# Autodesk Inventor assembly: CH-0-01-GearBoxAssembly
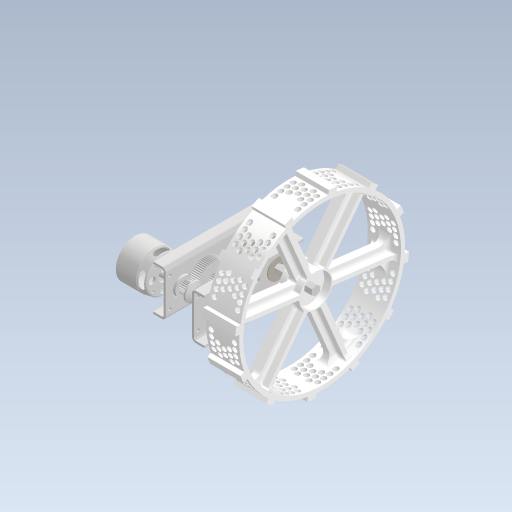
[picture p0: Inventor's stored thumbnail of the model, 512x512]
Saved by Autodesk Inventor 2023 (Build 270158000, 158)
## iProperties
Created: 2022-11-08
Part Number: CH-0-01-GearBoxAssembly
Document SubType Name: Assembly
Designer: Dave
Author: Dave
## Documents named in this file (13)
- C:\Users\Dave\Documents\GitHub\BehrendURCMechanical\CAD\Chassis\GearBox\CH-0-01-GearBoxAssembly.iam
- C:\Users\Dave\Documents\GitHub\BehrendURCMechanical\CAD\Chassis\GearBox\CH-1-01-0.5HexBearing.ipt
- C:\Users\Dave\Documents\GitHub\BehrendURCMechanical\CAD\Chassis\GearBox\CH-1-01-0.25IDSmoothBoreBearing.ipt
- C:\Users\Dave\Documents\GitHub\BehrendURCMechanical\CAD\Chassis\GearBox\CH-1-01-20T_0.5x0.25BoreGear.ipt
- C:\Users\Dave\Documents\GitHub\BehrendURCMechanical\CAD\Chassis\GearBox\CH-1-01-20T_0.5x8mmBoreGear.ipt
- C:\Users\Dave\Documents\GitHub\BehrendURCMechanical\CAD\Chassis\GearBox\CH-1-01-60T_0.5x0.25BoreGear.ipt
- C:\Users\Dave\Documents\GitHub\BehrendURCMechanical\CAD\Chassis\GearBox\Ch-1-01-0.5x4.5HexShaft.ipt
- C:\Users\Dave\Documents\GitHub\BehrendURCMechanical\CAD\Chassis\GearBox\CH-1-01-0.25x1.875SmoothShaft.ipt
- C:\Users\Dave\Documents\GitHub\BehrendURCMechanical\CAD\Chassis\CH-1-03-6SpokeWheel.ipt
- C:\Users\Dave\Documents\GitHub\BehrendURCMechanical\CAD\Chassis\GearBox\Drive Motor Shaft Coupler.ipt
- C:\Users\Dave\Documents\GitHub\BehrendURCMechanical\CAD\Chassis\GearBox\Drive Motor.ipt
- C:\Users\Dave\Documents\GitHub\BehrendURCMechanical\CAD\Chassis\GearBox\CH-1-01-GearboxHousingMotorSide.ipt
- C:\Users\Dave\Documents\GitHub\BehrendURCMechanical\CAD\Chassis\GearBox\CH-1-01-GearboxHousingWheelSide.ipt
## Components (20 placed, 12 different names)
1. CH-1-01-0.5HexBearing:1 — Mate:23, Flush:6, Mate:29, Insert:4, Mate:37
2. CH-1-01-0.5HexBearing:2 — Mate:21, Mate:23, Flush:8, Flush:9, Flush:12, Mate:26, Mate:27, Mate:33, Insert:3
3. CH-1-01-0.25IDSmoothBoreBearing:1 — Mate:18, Flush:9, Flush:11, Mate:25
4. CH-1-01-0.25IDSmoothBoreBearing:2 — Mate:17, Flush:8, Flush:10, Mate:24, Mate:35
5. CH-1-01-0.25IDSmoothBoreBearing:3 — Mate:19, Flush:6, Flush:7
6. CH-1-01-0.25IDSmoothBoreBearing:4 — Mate:16, Flush:7, Mate:36
7. CH-1-01-20T_0.5x0.25BoreGear:1 — Mate:4, Mate:5, Flush:3, Mate:6, Mate:16, Mate:31, Rotation:6
8. CH-1-01-20T_0.5x0.25BoreGear:2 — Mate:7, Mate:8, Mate:10, Mate:19, Angle:16
9. CH-1-01-20T_0.5x8mmBoreGear:1 — Mate:1, Flush:1, Flush:2, Mate:2, Rotation:1, Angle:2, Insert:1
10. CH-1-01-60T_0.5x0.25BoreGear:1 — Flush:3, Mate:6, Mate:7, Mate:8, Mate:18, Rotation:6, Angle:16, Mate:34
11. CH-1-01-60T_0.5x0.25BoreGear:2 — Flush:2, Mate:2, Mate:3, Mate:4, Mate:5, Mate:17, Mate:21, Rotation:1, Mate:31
12. Ch-1-01-0.5x4.5HexShaft:1 — Flush:12, Mate:26, Mate:27, Flush:14, Mate:30
13. CH-1-01-0.25x1.875SmoothShaft:1 — Flush:10, Mate:24
14. CH-1-01-0.25x1.875SmoothShaft:2 — Flush:11, Mate:25
15. CH-1-03-6SpokeWheel:1 — Mate:29, Flush:14, Mate:30
16. CH-1-01-60T_0.5x0.25BoreGear:3 — Mate:33, Mate:34, Mate:37
17. Drive Motor Shaft Coupler:1 — Insert:1, Insert:2
18. Drive Motor:1 — Insert:2
19. CH-1-01-GearboxHousingMotorSide:1 — Insert:3, Mate:35
20. CH-1-01-GearboxHousingWheelSide:1 — Insert:4, Mate:36
## Relationships (47: Mate 27, Flush 12, Insert 4, RelateRotation 2, Angle 2)
- Mate:1: CH-1-01-20T_0.5x8mmBoreGear:1
- Flush:1: CH-1-01-20T_0.5x8mmBoreGear:1
- Flush:2: CH-1-01-20T_0.5x8mmBoreGear:1 ↔ CH-1-01-60T_0.5x0.25BoreGear:2
- Mate:2 (31.75 mm): CH-1-01-20T_0.5x8mmBoreGear:1 ↔ CH-1-01-60T_0.5x0.25BoreGear:2
- Mate:3: CH-1-01-60T_0.5x0.25BoreGear:2
- Mate:4: CH-1-01-20T_0.5x0.25BoreGear:1 ↔ CH-1-01-60T_0.5x0.25BoreGear:2
- Mate:5: CH-1-01-20T_0.5x0.25BoreGear:1 ↔ CH-1-01-60T_0.5x0.25BoreGear:2
- Flush:3: CH-1-01-20T_0.5x0.25BoreGear:1 ↔ CH-1-01-60T_0.5x0.25BoreGear:1
- Mate:6 (31.75 mm): CH-1-01-20T_0.5x0.25BoreGear:1 ↔ CH-1-01-60T_0.5x0.25BoreGear:1
- Mate:7: CH-1-01-20T_0.5x0.25BoreGear:2 ↔ CH-1-01-60T_0.5x0.25BoreGear:1
- Mate:8: CH-1-01-20T_0.5x0.25BoreGear:2 ↔ CH-1-01-60T_0.5x0.25BoreGear:1
- Flush:5
- Mate:10: CH-1-01-20T_0.5x0.25BoreGear:2
- Mate:16: CH-1-01-0.25IDSmoothBoreBearing:4 ↔ CH-1-01-20T_0.5x0.25BoreGear:1
- Mate:17: CH-1-01-0.25IDSmoothBoreBearing:2 ↔ CH-1-01-60T_0.5x0.25BoreGear:2
- Mate:18: CH-1-01-0.25IDSmoothBoreBearing:1 ↔ CH-1-01-60T_0.5x0.25BoreGear:1
- Mate:19: CH-1-01-0.25IDSmoothBoreBearing:3 ↔ CH-1-01-20T_0.5x0.25BoreGear:2
- Mate:21: CH-1-01-0.5HexBearing:2 ↔ CH-1-01-60T_0.5x0.25BoreGear:2
- Mate:23: CH-1-01-0.5HexBearing:1 ↔ CH-1-01-0.5HexBearing:2
- Flush:6: CH-1-01-0.5HexBearing:1 ↔ CH-1-01-0.25IDSmoothBoreBearing:3
- Flush:7: CH-1-01-0.25IDSmoothBoreBearing:3 ↔ CH-1-01-0.25IDSmoothBoreBearing:4
- Flush:8: CH-1-01-0.5HexBearing:2 ↔ CH-1-01-0.25IDSmoothBoreBearing:2
- Flush:9: CH-1-01-0.5HexBearing:2 ↔ CH-1-01-0.25IDSmoothBoreBearing:1
- Flush:10: CH-1-01-0.25IDSmoothBoreBearing:2 ↔ CH-1-01-0.25x1.875SmoothShaft:1
- Mate:24: CH-1-01-0.25IDSmoothBoreBearing:2 ↔ CH-1-01-0.25x1.875SmoothShaft:1
- Flush:11: CH-1-01-0.25IDSmoothBoreBearing:1 ↔ CH-1-01-0.25x1.875SmoothShaft:2
- Mate:25: CH-1-01-0.25IDSmoothBoreBearing:1 ↔ CH-1-01-0.25x1.875SmoothShaft:2
- Flush:12: CH-1-01-0.5HexBearing:2 ↔ Ch-1-01-0.5x4.5HexShaft:1
- Mate:26: CH-1-01-0.5HexBearing:2 ↔ Ch-1-01-0.5x4.5HexShaft:1
- Mate:27: CH-1-01-0.5HexBearing:2 ↔ Ch-1-01-0.5x4.5HexShaft:1
- Mate:29: CH-1-01-0.5HexBearing:1 ↔ CH-1-03-6SpokeWheel:1
- Flush:14: Ch-1-01-0.5x4.5HexShaft:1 ↔ CH-1-03-6SpokeWheel:1
- Mate:30: Ch-1-01-0.5x4.5HexShaft:1 ↔ CH-1-03-6SpokeWheel:1
- Rotation:1 [RelateRotation] (0.3333 ul): CH-1-01-20T_0.5x8mmBoreGear:1 ↔ CH-1-01-60T_0.5x0.25BoreGear:2
- Angle:2 (926 deg): CH-1-01-20T_0.5x8mmBoreGear:1
- Mate:31: CH-1-01-20T_0.5x0.25BoreGear:1 ↔ CH-1-01-60T_0.5x0.25BoreGear:2
- Rotation:6 [RelateRotation] (0.3333 ul): CH-1-01-20T_0.5x0.25BoreGear:1 ↔ CH-1-01-60T_0.5x0.25BoreGear:1
- Angle:16 (0 deg): CH-1-01-20T_0.5x0.25BoreGear:2 ↔ CH-1-01-60T_0.5x0.25BoreGear:1
- Mate:33: CH-1-01-0.5HexBearing:2 ↔ CH-1-01-60T_0.5x0.25BoreGear:3
- Mate:34: CH-1-01-60T_0.5x0.25BoreGear:1 ↔ CH-1-01-60T_0.5x0.25BoreGear:3
- Insert:1: CH-1-01-20T_0.5x8mmBoreGear:1 ↔ Drive Motor Shaft Coupler:1
- Insert:2 (12.7 mm): Drive Motor Shaft Coupler:1 ↔ Drive Motor:1
- Insert:3: CH-1-01-0.5HexBearing:2 ↔ CH-1-01-GearboxHousingMotorSide:1
- Mate:35: CH-1-01-0.25IDSmoothBoreBearing:2 ↔ CH-1-01-GearboxHousingMotorSide:1
- Insert:4: CH-1-01-0.5HexBearing:1 ↔ CH-1-01-GearboxHousingWheelSide:1
- Mate:36: CH-1-01-0.25IDSmoothBoreBearing:4 ↔ CH-1-01-GearboxHousingWheelSide:1
- Mate:37 (2.54 mm): CH-1-01-0.5HexBearing:1 ↔ CH-1-01-60T_0.5x0.25BoreGear:3
